# Autodesk Inventor assembly: Assembly
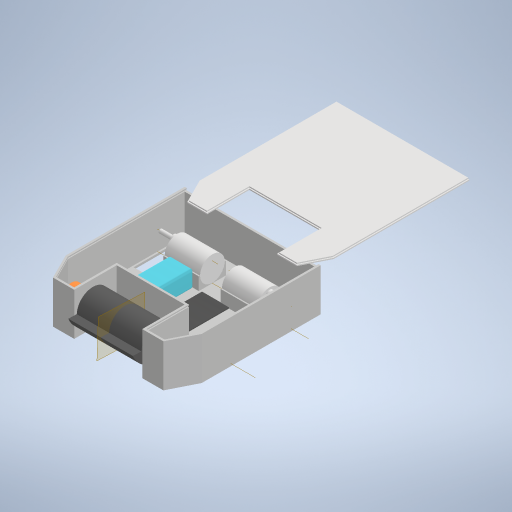
[picture p0: Inventor's stored thumbnail of the model, 512x512]
Saved by Autodesk Inventor 2024 (Build 280153000, 153)
## iProperties
Created: 2023-10-18
Part Number: Assembly
Document SubType Name: Assembly
Designer: CJ110
Author: CJ110
## Documents named in this file (8)
- D:\GitHub\Vault-1\CAD\WCRL\V1\Bot Assembly.iam
- D:\GitHub\Vault-1\CAD\WCRL\V1\Bot v1 bottom.ipt
- D:\GitHub\Vault-1\CAD\WCRL\V1\PCB.ipt
- D:\GitHub\Vault-1\CAD\WCRL\V1\LiPo.ipt
- D:\GitHub\Vault-1\CAD\WCRL\V1\Drum.ipt
- D:\GitHub\Vault-1\CAD\WCRL\V1\Bot v1 top.ipt
- D:\GitHub\Vault-1\CAD\WCRL\V1\Brushless 2622 2600KV.ipt
- D:\GitHub\Vault-1\CAD\WCRL\V1\DC 12V 200RPM.ipt
## Components (8 placed, 7 different names)
1. Bot v1 bottom:1 — Mate:5, Mate:6, Mate:11, Mate:16, Mate:18, Mate:19, Mate:20, Flush:1, Flush:23, Mate:24, Mate:25, Mate:26, Mate:27
2. PCB:1 — Mate:5
3. LiPo:2 — Mate:6
4. Drum:1 — Mate:11, Mate:23
5. Bot v1 top:1 — Mate:16, Mate:18
6. Brushless 2622 2600KV:1 — Mate:19, Mate:20, Mate:23
7. DC 12V 200RPM:1 — Flush:1, Mate:24, Mate:26
8. DC 12V 200RPM:2 — Flush:23, Mate:25, Mate:27
## Relationships (14: Mate 12, Flush 2)
- Mate:5: Bot v1 bottom:1 ↔ PCB:1
- Mate:6: Bot v1 bottom:1 ↔ LiPo:2
- Mate:11: Bot v1 bottom:1 ↔ Drum:1
- Mate:16: Bot v1 bottom:1 ↔ Bot v1 top:1
- Mate:18: Bot v1 bottom:1 ↔ Bot v1 top:1
- Mate:19: Bot v1 bottom:1 ↔ Brushless 2622 2600KV:1
- Mate:20: Bot v1 bottom:1 ↔ Brushless 2622 2600KV:1
- Flush:1: Bot v1 bottom:1 ↔ DC 12V 200RPM:1
- Flush:23: Bot v1 bottom:1 ↔ DC 12V 200RPM:2
- Mate:23: Drum:1 ↔ Brushless 2622 2600KV:1
- Mate:24: Bot v1 bottom:1 ↔ DC 12V 200RPM:1
- Mate:25: Bot v1 bottom:1 ↔ DC 12V 200RPM:2
- Mate:26: Bot v1 bottom:1 ↔ DC 12V 200RPM:1
- Mate:27: Bot v1 bottom:1 ↔ DC 12V 200RPM:2
